# Autodesk Inventor assembly: LIBS分光系
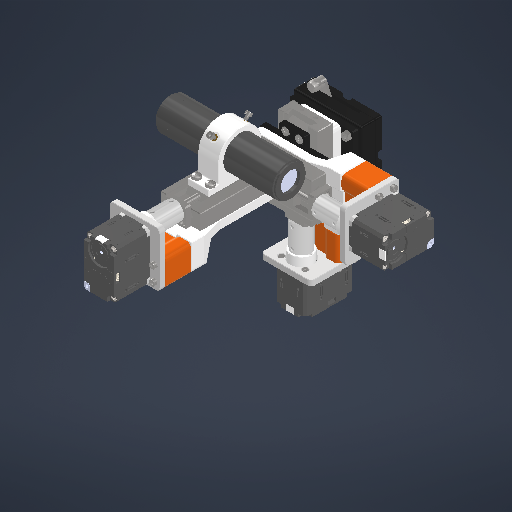
[picture p0: Inventor's stored thumbnail of the model, 512x512]
Saved by Autodesk Inventor 2026 (Build 300175050, 175E)
## iProperties
Created: 2025-07-15
Part Number: LIBS分光系
Document SubType Name: Assembly
Designer: jin20
Author: jin20
## Documents named in this file (4)
- C:\Users\jin20\Documents\装置CAD\RamanSystem\LIBS分光系.iam
- C:\Users\jin20\Documents\装置CAD\RamanSystem\Stage\マグネットベース.ipt
- C:\Users\jin20\Documents\装置CAD\PIHTI\LIBS\XL430-bracket.iam
- C:\Users\jin20\Documents\装置CAD\RamanSystem\Optics\チューブレンズ_縮尺変更.ipt
## Components (3 placed, 3 different names)
1. マグネットベース:1 — 挿入:1, 挿入:2, 挿入:3, 挿入:4
2. XL430-bracket:1 [sub-assembly] — 挿入:1, 挿入:2, 挿入:3, 挿入:4, 挿入:5
3. チューブレンズ_縮尺変更:1 — 挿入:5
## Relationships (5: Insert 5)
- 挿入:1 [Insert]: マグネットベース:1 ↔ XL430-bracket:1
- 挿入:2 [Insert]: マグネットベース:1 ↔ XL430-bracket:1
- 挿入:3 [Insert]: マグネットベース:1 ↔ XL430-bracket:1
- 挿入:4 [Insert]: マグネットベース:1 ↔ XL430-bracket:1
- 挿入:5 [Insert] (-45 mm): XL430-bracket:1 ↔ チューブレンズ_縮尺変更:1
